# Autodesk Inventor assembly: leftSide
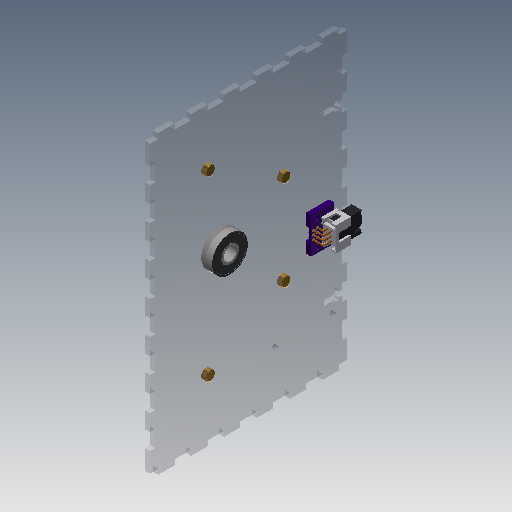
[picture p0: Inventor's stored thumbnail of the model, 512x512]
Saved by Autodesk Inventor 2018 (Build 220112000, 112)
## iProperties
Created: 2016-08-27
Part Number: leftSide
Document SubType Name: Assembly
Designer: sawaiz
Author: sawaiz
## Documents named in this file (5)
- C:\Users\sawaiz\OneDrive\projects\splitFlapDisplay\frame\leftSide.iam
- C:\Users\sawaiz\OneDrive\projects\splitFlapDisplay\frame\leftSide.ipt
- C:\Users\sawaiz\OneDrive\projects\splitFlapDisplay\frame\magnet.ipt
- C:\Users\sawaiz\OneDrive\projects\splitFlapDisplay\frame\608RS.ipt
- C:\Users\sawaiz\OneDrive\projects\splitFlapDisplay\electronics\cad\spring\spring.iam
## Components (7 placed, 4 different names)
1. leftSide:1 — Mate:1, Mate:2, Mate:3, Mate:4, Mate:5, Flush:4, Flush:5, Mate:6, Mate:7, Mate:8
2. magnet:1 — Mate:1, Flush:1, Flush:3, Flush:4
3. magnet:2 — Mate:4, Flush:1
4. magnet:3 — Mate:3, Flush:2
5. magnet:4 — Mate:2, Flush:2, Flush:3
6. 608RS:1 — Mate:5, Flush:5
7. spring:1 [sub-assembly] — Mate:6, Mate:7, Mate:8
## Relationships (13: Mate 8, Flush 5)
- Mate:1: leftSide:1 ↔ magnet:1
- Mate:2: leftSide:1 ↔ magnet:4
- Mate:3: leftSide:1 ↔ magnet:3
- Mate:4: leftSide:1 ↔ magnet:2
- Mate:5: leftSide:1 ↔ 608RS:1
- Flush:1: magnet:1 ↔ magnet:2
- Flush:2: magnet:3 ↔ magnet:4
- Flush:3: magnet:1 ↔ magnet:4
- Flush:4: leftSide:1 ↔ magnet:1
- Flush:5: leftSide:1 ↔ 608RS:1
- Mate:6: leftSide:1 ↔ spring:1
- Mate:7: leftSide:1 ↔ spring:1
- Mate:8: leftSide:1 ↔ spring:1
